# Autodesk Inventor assembly: Front Board Assembly
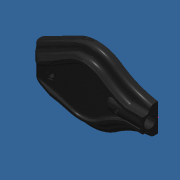
[picture p0: Inventor's stored thumbnail of the model, 180x180]
Saved by Autodesk Inventor 2018 (Build 220112000, 112)
## iProperties
Created: 2018-04-07
Part Number: Front Board Assembly
Document SubType Name: Assembly
Designer: Cole
Author: Cole
## Documents named in this file (3)
- D:\Cole\Documents\GitHub\SchoolCAD\ReverseEngineering\Front Board Assembly.iam
- D:\Cole\Documents\GitHub\SchoolCAD\ReverseEngineering\Front Board Cover.ipt
- D:\Cole\Documents\GitHub\SchoolCAD\ReverseEngineering\Front Board.ipt
## Components (2 placed, 2 different names)
1. Front Board Cover:1 — Mate:1, Mate:2
2. Front Board:1 — Mate:1, Mate:2
## Relationships (2: Mate 2)
- Mate:1: Front Board Cover:1 ↔ Front Board:1
- Mate:2: Front Board Cover:1 ↔ Front Board:1
